# Autodesk Inventor assembly: Assembly8
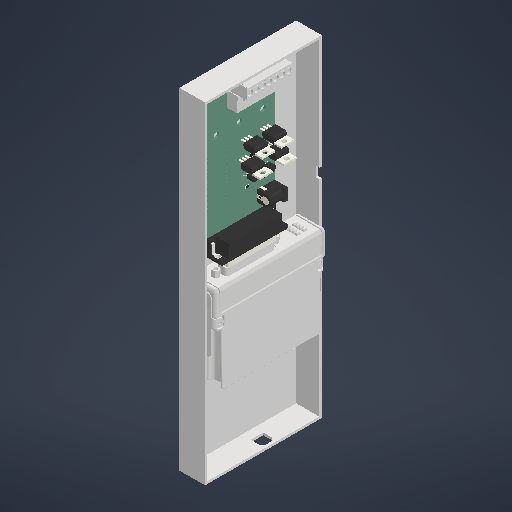
[picture p0: Inventor's stored thumbnail of the model, 512x512]
Saved by Autodesk Inventor 2027 (Build 310192000, 192)
## iProperties
Created: 2026-05-11
Part Number: Assembly8
Document SubType Name: Assembly
Designer: giese
Author: giese
## Documents named in this file (4)
- C:\Users\giese\OneDrive\Documents\GitHub\Biphasic-data-acquisition-system\DAQ_design\Assisi\v0.2.1\CAD\Assembly9.iam
- C:\Users\giese\OneDrive\Documents\Work\cdaq\cdaq.ipt
- C:\Users\giese\OneDrive\Documents\GitHub\Biphasic-data-acquisition-system\DAQ_design\Assisi\v0.2.1\EDA\assisi_v0.2.1\assisi_v0.2.1.ipt
- C:\Users\giese\OneDrive\Documents\GitHub\Biphasic-data-acquisition-system\DAQ_design\Assisi\v0.2.1\CAD\cDAQ_Bottom_Box6\cDAQ_Bottom_Box6.ipt
## Components (3 placed, 3 different names)
1. cdaq:1 — Mate:1
2. assisi_v0.2.1:1 — Mate:2
3. cDAQ_Bottom_Box6:1 — Mate:1, Mate:2
## Relationships (2: Mate 2)
- Mate:1: cdaq:1 ↔ cDAQ_Bottom_Box6:1
- Mate:2: assisi_v0.2.1:1 ↔ cDAQ_Bottom_Box6:1
